# Autodesk Inventor assembly: 110033226_iam_12_船屋
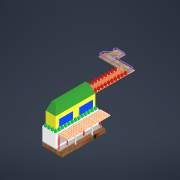
[picture p0: Inventor's stored thumbnail of the model, 180x180]
Saved by Autodesk Inventor 2022 (Build 260153000, 153)
## iProperties
Created: 2022-06-28
Part Number: 110033226_iam_12_船屋
Document SubType Name: Assembly
Designer: User
Author: User
## Documents named in this file (6)
- D:\D-disk\pomelo\大一\下學期\機械設計製圖\1100332260_LEGOproj_沒有公主城堡\110033226_iam_12_船屋.iam
- D:\D-disk\pomelo\大一\下學期\機械設計製圖\1100332260_LEGOproj_沒有公主城堡\110033226_ipt_47_船屋基地.ipt
- D:\D-disk\pomelo\大一\下學期\機械設計製圖\1100332260_LEGOproj_沒有公主城堡\110033226_ipt_48_船屋梁架.ipt
- D:\D-disk\pomelo\大一\下學期\機械設計製圖\1100332260_LEGOproj_沒有公主城堡\110033226_ipt_49_船屋主體.ipt
- D:\D-disk\pomelo\大一\下學期\機械設計製圖\1100332260_LEGOproj_沒有公主城堡\110033226_ipt_50_船屋圓柱.ipt
- D:\D-disk\pomelo\大一\下學期\機械設計製圖\1100332260_LEGOproj_沒有公主城堡\110033226_ipt_21_柵欄.ipt
## Components (73 placed, 5 different names)
1. 110033226_ipt_48_船屋梁架:1 — 貼合:4, 貼合:5, 貼合:7
2. 110033226_ipt_49_船屋主體:1 — 貼合:6, 貼合:7, 貼合:11, 貼合:12, 貼合:13, 貼合:14, 貼合:15, 貼合:16, 貼合:17, 貼合:18, 貼合:19, 貼合:20, 貼合:21, 貼合:22, 貼合:23, 貼合:24, 貼合:25, 貼合:26, 貼合:27, 貼合:28, 貼合:29, 貼合:30, 貼合:31, 貼合:32, 貼合:33, 貼合:34
3. 110033226_ipt_21_柵欄:32 — 貼合:27, 貼合:28, 貼合:29, 角度:1
4. 110033226_ipt_47_船屋基地:1 — 貼合:1, 貼合:2, 貼合:3
5. 110033226_ipt_47_船屋基地:2 — 貼合:4, 貼合:5, 貼合:6, 貼合:8, 貼合:9, 貼合:10, 貼合:13, 貼合:14
6. 110033226_ipt_50_船屋圓柱:1 — 貼合:8, 貼合:9, 貼合:10
7. 110033226_ipt_50_船屋圓柱:2
8. 110033226_ipt_21_柵欄:1 — 貼合:11, 貼合:12
9. 110033226_ipt_21_柵欄:2
10. 110033226_ipt_21_柵欄:3
11. 110033226_ipt_21_柵欄:4
12. 110033226_ipt_21_柵欄:5
13. 110033226_ipt_21_柵欄:6
14. 110033226_ipt_21_柵欄:7
15. 110033226_ipt_21_柵欄:8
16. 110033226_ipt_21_柵欄:9
17. 110033226_ipt_21_柵欄:10
18. 110033226_ipt_21_柵欄:11
19. 110033226_ipt_21_柵欄:12
20. 110033226_ipt_21_柵欄:13
21. 110033226_ipt_21_柵欄:14 — 貼合:15, 貼合:16, 貼合:17
22. 110033226_ipt_21_柵欄:15
23. 110033226_ipt_21_柵欄:16
24. 110033226_ipt_21_柵欄:17
25. 110033226_ipt_21_柵欄:18
26. 110033226_ipt_21_柵欄:19
27. 110033226_ipt_21_柵欄:21 — 貼合:18, 貼合:19, 貼合:20
28. 110033226_ipt_21_柵欄:23
29. 110033226_ipt_21_柵欄:22 — 貼合:21, 貼合:22, 貼合:23
30. 110033226_ipt_21_柵欄:24
31. 110033226_ipt_21_柵欄:25
32. 110033226_ipt_21_柵欄:26
33. 110033226_ipt_21_柵欄:27
34. 110033226_ipt_21_柵欄:20 — 貼合:24, 貼合:25, 貼合:26
35. 110033226_ipt_21_柵欄:28
36. 110033226_ipt_21_柵欄:29
37. 110033226_ipt_21_柵欄:30
38. 110033226_ipt_21_柵欄:31 — 貼合:30, 貼合:31, 角度:1
39. 110033226_ipt_21_柵欄:33
40. 110033226_ipt_21_柵欄:34
41. 110033226_ipt_21_柵欄:35
42. 110033226_ipt_21_柵欄:36
43. 110033226_ipt_21_柵欄:37
44. 110033226_ipt_21_柵欄:38
45. 110033226_ipt_21_柵欄:39
46. 110033226_ipt_21_柵欄:40
47. 110033226_ipt_21_柵欄:41
48. 110033226_ipt_21_柵欄:42
49. 110033226_ipt_21_柵欄:43
50. 110033226_ipt_21_柵欄:44
51. 110033226_ipt_21_柵欄:45
52. 110033226_ipt_21_柵欄:46
53. 110033226_ipt_21_柵欄:47
54. 110033226_ipt_21_柵欄:48
55. 110033226_ipt_21_柵欄:49 — 貼合:32, 貼合:33, 貼合:34
56. 110033226_ipt_21_柵欄:50
57. 110033226_ipt_21_柵欄:51
58. 110033226_ipt_21_柵欄:52
59. 110033226_ipt_21_柵欄:53
60. 110033226_ipt_21_柵欄:54
61. 110033226_ipt_21_柵欄:55
62. 110033226_ipt_21_柵欄:56
63. 110033226_ipt_21_柵欄:57
64. 110033226_ipt_21_柵欄:58
65. 110033226_ipt_21_柵欄:59
66. 110033226_ipt_21_柵欄:60
67. 110033226_ipt_21_柵欄:61
68. 110033226_ipt_21_柵欄:62
69. 110033226_ipt_21_柵欄:63
70. 110033226_ipt_21_柵欄:64
71. 110033226_ipt_21_柵欄:65
72. 110033226_ipt_21_柵欄:66
73. 110033226_ipt_21_柵欄:67
## Component patterns: (2 elements, first: 110033226_ipt_47_船屋基地:1), (2 elements, first: 110033226_ipt_50_船屋圓柱:1), (13 elements, first: 110033226_ipt_21_柵欄:1), (6 elements, first: 110033226_ipt_21_柵欄:14), (2 elements, first: 110033226_ipt_21_柵欄:21), (5 elements, first: 110033226_ipt_21_柵欄:22), (4 elements, first: 110033226_ipt_21_柵欄:20), (17 elements, first: 110033226_ipt_21_柵欄:31), (19 elements, first: 110033226_ipt_21_柵欄:49)
## Relationships (35: Mate 34, Angle 1)
- 貼合:1 [Mate]: 110033226_ipt_47_船屋基地:1
- 貼合:2 [Mate]: 110033226_ipt_47_船屋基地:1
- 貼合:3 [Mate]: 110033226_ipt_47_船屋基地:1
- 貼合:4 [Mate]: 110033226_ipt_48_船屋梁架:1 ↔ 110033226_ipt_47_船屋基地:2
- 貼合:5 [Mate]: 110033226_ipt_48_船屋梁架:1 ↔ 110033226_ipt_47_船屋基地:2
- 貼合:6 [Mate]: 110033226_ipt_49_船屋主體:1 ↔ 110033226_ipt_47_船屋基地:2
- 貼合:7 [Mate]: 110033226_ipt_48_船屋梁架:1 ↔ 110033226_ipt_49_船屋主體:1
- 貼合:8 [Mate]: 110033226_ipt_47_船屋基地:2 ↔ 110033226_ipt_50_船屋圓柱:1
- 貼合:9 [Mate]: 110033226_ipt_47_船屋基地:2 ↔ 110033226_ipt_50_船屋圓柱:1
- 貼合:10 [Mate]: 110033226_ipt_47_船屋基地:2 ↔ 110033226_ipt_50_船屋圓柱:1
- 貼合:11 [Mate]: 110033226_ipt_49_船屋主體:1 ↔ 110033226_ipt_21_柵欄:1
- 貼合:12 [Mate]: 110033226_ipt_49_船屋主體:1 ↔ 110033226_ipt_21_柵欄:1
- 貼合:13 [Mate]: 110033226_ipt_49_船屋主體:1 ↔ 110033226_ipt_47_船屋基地:2
- 貼合:14 [Mate]: 110033226_ipt_49_船屋主體:1 ↔ 110033226_ipt_47_船屋基地:2
- 貼合:15 [Mate]: 110033226_ipt_49_船屋主體:1 ↔ 110033226_ipt_21_柵欄:14
- 貼合:16 [Mate]: 110033226_ipt_49_船屋主體:1 ↔ 110033226_ipt_21_柵欄:14
- 貼合:17 [Mate]: 110033226_ipt_49_船屋主體:1 ↔ 110033226_ipt_21_柵欄:14
- 貼合:18 [Mate]: 110033226_ipt_49_船屋主體:1 ↔ 110033226_ipt_21_柵欄:21
- 貼合:19 [Mate]: 110033226_ipt_49_船屋主體:1 ↔ 110033226_ipt_21_柵欄:21
- 貼合:20 [Mate]: 110033226_ipt_49_船屋主體:1 ↔ 110033226_ipt_21_柵欄:21
- 貼合:21 [Mate]: 110033226_ipt_49_船屋主體:1 ↔ 110033226_ipt_21_柵欄:22
- 貼合:22 [Mate]: 110033226_ipt_49_船屋主體:1 ↔ 110033226_ipt_21_柵欄:22
- 貼合:23 [Mate]: 110033226_ipt_49_船屋主體:1 ↔ 110033226_ipt_21_柵欄:22
- 貼合:24 [Mate]: 110033226_ipt_49_船屋主體:1 ↔ 110033226_ipt_21_柵欄:20
- 貼合:25 [Mate]: 110033226_ipt_49_船屋主體:1 ↔ 110033226_ipt_21_柵欄:20
- 貼合:26 [Mate]: 110033226_ipt_49_船屋主體:1 ↔ 110033226_ipt_21_柵欄:20
- 貼合:27 [Mate]: 110033226_ipt_49_船屋主體:1 ↔ 110033226_ipt_21_柵欄:32
- 貼合:28 [Mate]: 110033226_ipt_49_船屋主體:1 ↔ 110033226_ipt_21_柵欄:32
- 貼合:29 [Mate]: 110033226_ipt_49_船屋主體:1 ↔ 110033226_ipt_21_柵欄:32
- 貼合:30 [Mate]: 110033226_ipt_49_船屋主體:1 ↔ 110033226_ipt_21_柵欄:31
- 貼合:31 [Mate]: 110033226_ipt_49_船屋主體:1 ↔ 110033226_ipt_21_柵欄:31
- 角度:1 [Angle] (90 deg): 110033226_ipt_21_柵欄:32 ↔ 110033226_ipt_21_柵欄:31
- 貼合:32 [Mate]: 110033226_ipt_49_船屋主體:1 ↔ 110033226_ipt_21_柵欄:49
- 貼合:33 [Mate]: 110033226_ipt_49_船屋主體:1 ↔ 110033226_ipt_21_柵欄:49
- 貼合:34 [Mate]: 110033226_ipt_49_船屋主體:1 ↔ 110033226_ipt_21_柵欄:49
